# Autodesk Inventor assembly: tarot_5008_340kv_assy
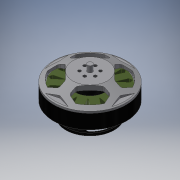
[picture p0: Inventor's stored thumbnail of the model, 180x180]
Saved by Autodesk Inventor 2019.4 (Build 234330000, 330)
## iProperties
Created: 2019-10-01
Part Number: tarot_5008_340kv_assy
Document SubType Name: Assembly
Designer: cdi
Author: cdi
## Documents named in this file (7)
- D:\SynologyDrive\workspace_inventor\2019_06_19.MT4008_actuator\tarot_5008_340kv\tarot_5008_340kv_assy.iam
- D:\SynologyDrive\workspace_inventor\2019_06_19.MT4008_actuator\tarot_5008_340kv\housing0.ipt
- D:\SynologyDrive\workspace_inventor\2019_06_19.MT4008_actuator\tarot_5008_340kv\housing1.ipt
- D:\SynologyDrive\workspace_inventor\2019_06_19.MT4008_actuator\tarot_5008_340kv\arc_magnet_10_10_2.ipt
- D:\SynologyDrive\workspace_inventor\2019_06_19.MT4008_actuator\tarot_5008_340kv\stator.ipt
- D:\SynologyDrive\workspace_inventor\2019_06_19.MT4008_actuator\tarot_5008_340kv\core.ipt
- D:\SynologyDrive\workspace_inventor\2019_06_19.MT4008_actuator\tarot_5008_340kv\bearing_6_12_3.ipt
## Components (19 placed, 6 different names)
1. housing0:1 — Mate:1, Mate:3, Mate:5, Mate:7, Mate:8, Flush:3
2. housing1:1 — Mate:2, Mate:3, Mate:6
3. stator:1 — Mate:7, Flush:1, Flush:2
4. core:1 — Mate:8, Flush:2, Mate:9
5. bearing_6_12_3:1 — Mate:9, Flush:3
6. arc_magnet_10_10_2:1 — Mate:5, Mate:6, Angle:1
7. arc_magnet_10_10_2:2
8. arc_magnet_10_10_2:3
9. arc_magnet_10_10_2:4
10. arc_magnet_10_10_2:5 — Flush:1
11. arc_magnet_10_10_2:6
12. arc_magnet_10_10_2:7
13. arc_magnet_10_10_2:8
14. arc_magnet_10_10_2:9
15. arc_magnet_10_10_2:10
16. arc_magnet_10_10_2:11
17. arc_magnet_10_10_2:12
18. arc_magnet_10_10_2:13
19. arc_magnet_10_10_2:14
## Component patterns: (14 elements, first: arc_magnet_10_10_2:1)
## Relationships (12: Mate 8, Flush 3, Angle 1)
- Mate:1: housing0:1
- Mate:2: housing1:1
- Mate:3: housing0:1 ↔ housing1:1
- Mate:5: housing0:1 ↔ arc_magnet_10_10_2:1
- Mate:6: housing1:1 ↔ arc_magnet_10_10_2:1
- Angle:1 (0 deg): arc_magnet_10_10_2:1
- Mate:7: housing0:1 ↔ stator:1
- Flush:1: stator:1 ↔ arc_magnet_10_10_2:5
- Mate:8: housing0:1 ↔ core:1
- Flush:2: stator:1 ↔ core:1
- Mate:9: core:1 ↔ bearing_6_12_3:1
- Flush:3: housing0:1 ↔ bearing_6_12_3:1
